# Autodesk Inventor assembly: assembly
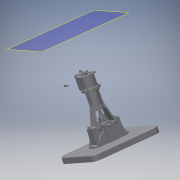
[picture p0: Inventor's stored thumbnail of the model, 180x180]
Saved by Autodesk Inventor 2017 (Build 210142000, 142)
## iProperties
Created: 2018-11-19
Part Number: assembly
Document SubType Name: Assembly
Designer: Arman Grewal
Author: Arman Grewal
## Documents named in this file (33)
- C:\Users\Arman Grewal\Desktop\Engine\assembly.iam
- C:\Users\Arman Grewal\Desktop\Engine\Piston.ipt
- C:\Users\Arman Grewal\Desktop\Engine\Piston Rod.ipt
- C:\Users\Arman Grewal\Documents\Inventor\Content Center Files\R2017\en-US\DIN 934\DIN 934 - M4 x 0.7.ipt
- C:\Users\Arman Grewal\Desktop\Engine\Crosshead.ipt
- C:\Users\Arman Grewal\Desktop\Engine\Crankrod.ipt
- C:\Users\Arman Grewal\Desktop\Engine\Crankrod Pin.ipt
- C:\Users\Arman Grewal\Desktop\Engine\Crankshaft Center Rod.ipt
- C:\Users\Arman Grewal\Desktop\Engine\Crankshaft outer rod.ipt
- C:\Users\Arman Grewal\Desktop\Engine\Crankshaft Counterweight.ipt
- C:\Users\Arman Grewal\Desktop\Engine\Vertical Steam Engine with Reverse Gear (anno 1830) Connecting Rod.ipt
- C:\Users\Arman Grewal\Desktop\Engine\Bearing Keeper.ipt
- C:\Users\Arman Grewal\Documents\Inventor\Content Center Files\R2017\en-US\DIN 84\DIN 84 - M3 x 20.ipt
- C:\Users\Arman Grewal\Desktop\Engine\Stand.ipt
- C:\Users\Arman Grewal\Desktop\Engine\Base cast f.ipt
- C:\Users\Arman Grewal\Documents\Inventor\Content Center Files\R2017\en-US\DIN 912\DIN 912 - M4 x 0.7 x 20 x 18.25.ipt
- C:\Users\Arman Grewal\Documents\Inventor\Content Center Files\R2017\en-US\DIN 6797  J\DIN 6797 - J 4.3.ipt
- C:\Users\Arman Grewal\Documents\Inventor\Content Center Files\R2017\en-US\DIN 6797  J\DIN 6797 - J 5.3.ipt
- C:\Users\Arman Grewal\Documents\Inventor\Content Center Files\R2017\en-US\DIN 934\DIN 934 - M5 x 0.8.ipt
- C:\Users\Arman Grewal\Desktop\Engine\Lower Base Bearing Holder.ipt
- C:\Users\Arman Grewal\Desktop\Engine\Upper Base Bearing Holder.ipt
- C:\Users\Arman Grewal\Documents\Inventor\Content Center Files\R2017\en-US\DIN 84\DIN 84 - M3 x 4.ipt
- C:\Users\Arman Grewal\Desktop\Engine\Standard.ipt
- C:\Users\Arman Grewal\Desktop\Engine\cylinder.ipt
- C:\Users\Arman Grewal\Documents\Inventor\Content Center Files\R2017\en-US\DIN 912\DIN 912 - M3 x 0.5 x 8 x 6.75.ipt
- C:\Users\Arman Grewal\Documents\Inventor\Content Center Files\R2017\en-US\DIN 128\DIN 128 - A3.5.ipt
- C:\Users\Arman Grewal\Desktop\Engine\Valve Plate.ipt
- C:\Users\Arman Grewal\Desktop\Engine\Steam Chest.ipt
- C:\Users\Arman Grewal\Desktop\Engine\Glands.ipt
- C:\Users\Arman Grewal\Desktop\Engine\Steam Chest Slide Valve Rod.ipt
- C:\Users\Arman Grewal\Desktop\Engine\Steam Chest Slide Valve.ipt
- C:\Users\Arman Grewal\Documents\Inventor\Content Center Files\R2017\en-US\DIN 84\DIN 84 - M2.5 x 10.ipt
- C:\Users\Arman Grewal\Documents\Inventor\Content Center Files\R2017\en-US\DIN 912\DIN 912 - M3 x 0.5 x 20 x 18.75.ipt
## Components (84 placed, 32 different names)
1. Piston:1 — Mate:1, Mate:2, Insert:1, Angle:2, Mate:56
2. Piston Rod:1 — Mate:1, Mate:2, Mate:3, Mate:4
3. DIN 934 - replaced by DIN EN 24032/28673/28674 M4:1 — Insert:1
4. Crosshead:1 — Mate:3, Mate:4, Mate:5, Mate:6
5. Crankrod:1 — Mate:5, Mate:6, Mate:7, Mate:8, Mate:9, Mate:10, Mate:11
6. Crankrod Pin:1 — Mate:7, Mate:8
7. Crankshaft Center Rod:1 — Mate:18, Mate:23, Mate:24, Mate:25, Mate:26
8. Crankshaft outer rod:1 — Mate:19, Mate:20, Mate:41
9. Crankshaft outer rod:2 — Mate:21, Mate:22
10. Vertical Steam Engine with Reverse Gear (anno 1830) Connecting Rod:1 — Mate:12, Mate:13, Mate:14, Mate:15, Mate:16, Mate:17
11. Vertical Steam Engine with Reverse Gear (anno 1830) Connecting Rod:2 — Mate:9, Mate:10, Mate:11, Mate:12, Mate:13, Mate:14, Mate:18, Mate:27
12. Bearing Keeper:1 — Mate:15, Mate:16, Mate:17, Insert:2, Insert:3
13. Crankshaft Counterweight:1 — Mate:21, Mate:22, Mate:25, Mate:26
14. Crankshaft Counterweight:2 — Mate:19, Mate:20, Mate:23, Mate:24, Mate:27, Mate:42
15. DIN 84 - replaced by DIN EN ISO 1207 M3 x 20:1 — Insert:2
16. DIN 84 - replaced by DIN EN ISO 1207 M3 x 20:2 — Insert:3
17. Stand:1 — Mate:28, Mate:29, Mate:30, Mate:32, Insert:8, Insert:9, Insert:10, Insert:11, Insert:20, Mate:36, Angle:1
18. Base cast f:1 — Mate:28, Mate:29, Mate:30, Insert:4, Insert:5, Insert:6, Insert:7, Mate:37, Flush:1, Mate:38, Mate:39, Flush:2, Mate:40, Mate:42, Mate:44, Mate:45, Mate:47, Mate:48, Mate:49, Mate:50, Mate:51, Mate:52
19. DIN 912 - replaced by DIN EN ISO 4762 M4 x 20:1 — Insert:4, Mate:31, Mate:33
20. DIN 912 - replaced by DIN EN ISO 4762 M4 x 20:2 — Insert:5
21. DIN 912 - replaced by DIN EN ISO 4762 M4 x 20:3 — Insert:6
22. DIN 912 - replaced by DIN EN ISO 4762 M4 x 20:4 — Insert:7, Mate:35
23. DIN 6797 J J 4.3:1 — Mate:31, Mate:32, Mate:34
24. DIN 6797 J J 5.3:1 — Insert:8, Insert:12, Insert:13, Insert:14, Insert:15, Insert:16, Insert:17, Insert:18, Insert:19
25. DIN 6797 J J 5.3:2 — Insert:9
26. DIN 6797 J J 5.3:3 — Insert:10
27. DIN 6797 J J 5.3:4 — Insert:11
28. DIN 934 - replaced by DIN EN 24032/28673/28674 M5:1 — Insert:12
29. DIN 934 - replaced by DIN EN 24032/28673/28674 M5:2 — Insert:13
30. DIN 934 - replaced by DIN EN 24032/28673/28674 M5:3 — Insert:14
31. DIN 934 - replaced by DIN EN 24032/28673/28674 M5:4 — Insert:15
32. DIN 934 - replaced by DIN EN 24032/28673/28674 M5:5 — Insert:16
33. DIN 934 - replaced by DIN EN 24032/28673/28674 M5:6 — Insert:17
34. DIN 934 - replaced by DIN EN 24032/28673/28674 M5:7 — Insert:18
35. DIN 934 - replaced by DIN EN 24032/28673/28674 M5:8 — Insert:19
36. DIN 934 - replaced by DIN EN 24032/28673/28674 M4:2 — Mate:33, Mate:34
37. DIN 934 - replaced by DIN EN 24032/28673/28674 M4:3 — Insert:20
38. DIN 934 - replaced by DIN EN 24032/28673/28674 M4:4 — Mate:35, Mate:36
39. Lower Base Bearing Holder:1 — Mate:37, Flush:1, Mate:38, Mate:41, Mate:46
40. Lower Base Bearing Holder:2 — Mate:39, Flush:2, Mate:40, Mate:43
41. Upper Base Bearing Holder:1 — Mate:46, Mate:47, Mate:48, Insert:21, Insert:22, Insert:23, Insert:24
42. Upper Base Bearing Holder:2 — Mate:43, Mate:44, Mate:45, Insert:25, Insert:26, Insert:27, Insert:28
43. DIN 84 - replaced by DIN EN ISO 1207 M3 x 4:1 — Insert:21
44. DIN 84 - replaced by DIN EN ISO 1207 M3 x 4:2 — Insert:22
45. DIN 84 - replaced by DIN EN ISO 1207 M3 x 4:3 — Insert:23
46. DIN 84 - replaced by DIN EN ISO 1207 M3 x 4:4 — Insert:24
47. DIN 84 - replaced by DIN EN ISO 1207 M3 x 4:5 — Insert:25
48. DIN 84 - replaced by DIN EN ISO 1207 M3 x 4:6 — Insert:26
49. DIN 84 - replaced by DIN EN ISO 1207 M3 x 4:7 — Insert:27
50. DIN 84 - replaced by DIN EN ISO 1207 M3 x 4:8 — Insert:28
51. Standard:1 — Mate:49, Mate:50, Mate:51, Mate:52, Mate:53, Mate:54, Mate:55, Insert:29, Insert:30, Insert:31, Insert:32, Insert:33, Insert:34, Insert:35, Insert:36, Insert:37, Insert:38, Insert:39, Insert:40, Insert:41, Insert:42, Insert:43, Insert:46
52. cylinder:1 — Mate:53, Angle:1, Mate:54, Mate:55, Angle:2, Mate:56, Mate:60, Mate:61, Mate:62
53. DIN 912 - replaced by DIN EN ISO 4762 M3 x 8:1 — Insert:29
54. DIN 912 - replaced by DIN EN ISO 4762 M3 x 8:2 — Insert:30
55. DIN 912 - replaced by DIN EN ISO 4762 M3 x 8:3 — Insert:31
56. DIN 912 - replaced by DIN EN ISO 4762 M3 x 8:4 — Insert:32
57. DIN 912 - replaced by DIN EN ISO 4762 M3 x 8:5 — Insert:33
58. DIN 912 - replaced by DIN EN ISO 4762 M3 x 8:6 — Insert:34
59. DIN 128 A3.5:1 — Insert:35
60. DIN 128 A3.5:2 — Insert:36, Insert:47
61. DIN 128 A3.5:3 — Insert:37, Insert:49
62. DIN 128 A3.5:4 — Insert:38, Insert:45
63. DIN 128 A3.5:5 — Insert:39, Insert:44
64. DIN 128 A3.5:6 — Insert:40, Insert:48
65. DIN 128 A3.5:7 — Insert:41, Insert:50
66. DIN 128 A3.5:8 — Insert:42
67. DIN 912 - replaced by DIN EN ISO 4762 M3 x 8:7 — Insert:43
68. DIN 912 - replaced by DIN EN ISO 4762 M3 x 8:8 — Insert:44
69. DIN 912 - replaced by DIN EN ISO 4762 M3 x 8:9 — Insert:45
70. DIN 912 - replaced by DIN EN ISO 4762 M3 x 8:10 — Insert:46
71. DIN 912 - replaced by DIN EN ISO 4762 M3 x 8:11 — Insert:47
72. DIN 912 - replaced by DIN EN ISO 4762 M3 x 8:12 — Insert:48
73. DIN 912 - replaced by DIN EN ISO 4762 M3 x 8:13 — Insert:49
74. DIN 912 - replaced by DIN EN ISO 4762 M3 x 8:14 — Insert:50
75. Valve Plate:1 — Mate:60, Mate:61, Mate:62, Mate:63, Mate:64, Mate:65
76. Steam Chest:1 — Mate:63, Mate:64, Mate:65, Mate:66, Mate:67, Mate:68, Mate:69, Mate:74
77. Glands:1 — Mate:66, Mate:67, Mate:68, Mate:69, Insert:67, Insert:68
78. Steam Chest Slide Valve Rod:1 — Mate:74, Mate:75, Mate:76, Mate:77, Mate:79
79. Steam Chest Slide Valve:1 — Mate:75, Mate:76, Mate:78, Mate:80
80. DIN 934 - replaced by DIN EN 24032/28673/28674 M4:5 — Mate:77, Mate:78
81. DIN 934 - replaced by DIN EN 24032/28673/28674 M4:6 — Mate:79, Mate:80
82. DIN 84 - replaced by DIN EN ISO 1207 M2.5 x 10:1 — Insert:67
83. DIN 84 - replaced by DIN EN ISO 1207 M2.5 x 10:2 — Insert:68
84. DIN 912 - replaced by DIN EN ISO 4762 M3 x 20:2
## Relationships (129: Mate 73, Insert 52, Flush 2, Angle 2)
- Mate:1: Piston:1 ↔ Piston Rod:1
- Mate:2: Piston:1 ↔ Piston Rod:1
- Insert:1: Piston:1 ↔ DIN 934 - replaced by DIN EN 24032/28673/28674 M4:1
- Mate:3: Piston Rod:1 ↔ Crosshead:1
- Mate:4 (-7.628 mm): Piston Rod:1 ↔ Crosshead:1
- Mate:5: Crosshead:1 ↔ Crankrod:1
- Mate:6: Crosshead:1 ↔ Crankrod:1
- Mate:7: Crankrod:1 ↔ Crankrod Pin:1
- Mate:8: Crankrod:1 ↔ Crankrod Pin:1
- Mate:9: Crankrod:1 ↔ Vertical Steam Engine with Reverse Gear (anno 1830) Connecting Rod:2
- Mate:10: Crankrod:1 ↔ Vertical Steam Engine with Reverse Gear (anno 1830) Connecting Rod:2
- Mate:11: Crankrod:1 ↔ Vertical Steam Engine with Reverse Gear (anno 1830) Connecting Rod:2
- Mate:12: Vertical Steam Engine with Reverse Gear (anno 1830) Connecting Rod:1 ↔ Vertical Steam Engine with Reverse Gear (anno 1830) Connecting Rod:2
- Mate:13: Vertical Steam Engine with Reverse Gear (anno 1830) Connecting Rod:1 ↔ Vertical Steam Engine with Reverse Gear (anno 1830) Connecting Rod:2
- Mate:14: Vertical Steam Engine with Reverse Gear (anno 1830) Connecting Rod:1 ↔ Vertical Steam Engine with Reverse Gear (anno 1830) Connecting Rod:2
- Mate:15: Vertical Steam Engine with Reverse Gear (anno 1830) Connecting Rod:1 ↔ Bearing Keeper:1
- Mate:16: Vertical Steam Engine with Reverse Gear (anno 1830) Connecting Rod:1 ↔ Bearing Keeper:1
- Mate:17: Vertical Steam Engine with Reverse Gear (anno 1830) Connecting Rod:1 ↔ Bearing Keeper:1
- Mate:18: Crankshaft Center Rod:1 ↔ Vertical Steam Engine with Reverse Gear (anno 1830) Connecting Rod:2
- Mate:19: Crankshaft outer rod:1 ↔ Crankshaft Counterweight:2
- Mate:20: Crankshaft outer rod:1 ↔ Crankshaft Counterweight:2
- Mate:21: Crankshaft outer rod:2 ↔ Crankshaft Counterweight:1
- Mate:22: Crankshaft outer rod:2 ↔ Crankshaft Counterweight:1
- Mate:23: Crankshaft Center Rod:1 ↔ Crankshaft Counterweight:2
- Mate:24: Crankshaft Center Rod:1 ↔ Crankshaft Counterweight:2
- Mate:25: Crankshaft Center Rod:1 ↔ Crankshaft Counterweight:1
- Mate:26: Crankshaft Center Rod:1 ↔ Crankshaft Counterweight:1
- Mate:27 (0.5 mm): Vertical Steam Engine with Reverse Gear (anno 1830) Connecting Rod:2 ↔ Crankshaft Counterweight:2
- Insert:2: Bearing Keeper:1 ↔ DIN 84 - replaced by DIN EN ISO 1207 M3 x 20:1
- Insert:3: Bearing Keeper:1 ↔ DIN 84 - replaced by DIN EN ISO 1207 M3 x 20:2
- Mate:28: Stand:1 ↔ Base cast f:1
- Mate:29: Stand:1 ↔ Base cast f:1
- Mate:30: Stand:1 ↔ Base cast f:1
- Insert:4: Base cast f:1 ↔ DIN 912 - replaced by DIN EN ISO 4762 M4 x 20:1
- Insert:5: Base cast f:1 ↔ DIN 912 - replaced by DIN EN ISO 4762 M4 x 20:2
- Insert:6: Base cast f:1 ↔ DIN 912 - replaced by DIN EN ISO 4762 M4 x 20:3
- Insert:7: Base cast f:1 ↔ DIN 912 - replaced by DIN EN ISO 4762 M4 x 20:4
- Mate:31: DIN 912 - replaced by DIN EN ISO 4762 M4 x 20:1 ↔ DIN 6797 J J 4.3:1
- Mate:32: Stand:1 ↔ DIN 6797 J J 4.3:1
- Insert:8: Stand:1 ↔ DIN 6797 J J 5.3:1
- Insert:9: Stand:1 ↔ DIN 6797 J J 5.3:2
- Insert:10: Stand:1 ↔ DIN 6797 J J 5.3:3
- Insert:11: Stand:1 ↔ DIN 6797 J J 5.3:4
- Insert:12: DIN 6797 J J 5.3:1 ↔ DIN 934 - replaced by DIN EN 24032/28673/28674 M5:1
- Insert:13: DIN 6797 J J 5.3:1 ↔ DIN 934 - replaced by DIN EN 24032/28673/28674 M5:2
- Insert:14: DIN 6797 J J 5.3:1 ↔ DIN 934 - replaced by DIN EN 24032/28673/28674 M5:3
- Insert:15: DIN 6797 J J 5.3:1 ↔ DIN 934 - replaced by DIN EN 24032/28673/28674 M5:4
- Insert:16: DIN 6797 J J 5.3:1 ↔ DIN 934 - replaced by DIN EN 24032/28673/28674 M5:5
- Insert:17: DIN 6797 J J 5.3:1 ↔ DIN 934 - replaced by DIN EN 24032/28673/28674 M5:6
- Insert:18: DIN 6797 J J 5.3:1 ↔ DIN 934 - replaced by DIN EN 24032/28673/28674 M5:7
- Insert:19: DIN 6797 J J 5.3:1 ↔ DIN 934 - replaced by DIN EN 24032/28673/28674 M5:8
- Mate:33: DIN 912 - replaced by DIN EN ISO 4762 M4 x 20:1 ↔ DIN 934 - replaced by DIN EN 24032/28673/28674 M4:2
- Mate:34: DIN 6797 J J 4.3:1 ↔ DIN 934 - replaced by DIN EN 24032/28673/28674 M4:2
- Insert:20: Stand:1 ↔ DIN 934 - replaced by DIN EN 24032/28673/28674 M4:3
- Mate:35: DIN 912 - replaced by DIN EN ISO 4762 M4 x 20:4 ↔ DIN 934 - replaced by DIN EN 24032/28673/28674 M4:4
- Mate:36: Stand:1 ↔ DIN 934 - replaced by DIN EN 24032/28673/28674 M4:4
- Mate:37: Base cast f:1 ↔ Lower Base Bearing Holder:1
- Flush:1: Base cast f:1 ↔ Lower Base Bearing Holder:1
- Mate:38: Base cast f:1 ↔ Lower Base Bearing Holder:1
- Mate:39: Base cast f:1 ↔ Lower Base Bearing Holder:2
- Flush:2: Base cast f:1 ↔ Lower Base Bearing Holder:2
- Mate:40: Base cast f:1 ↔ Lower Base Bearing Holder:2
- Mate:41: Crankshaft outer rod:1 ↔ Lower Base Bearing Holder:1
- Mate:42 (2.5 mm): Crankshaft Counterweight:2 ↔ Base cast f:1
- Mate:43: Lower Base Bearing Holder:2 ↔ Upper Base Bearing Holder:2
- Mate:44: Base cast f:1 ↔ Upper Base Bearing Holder:2
- Mate:45: Base cast f:1 ↔ Upper Base Bearing Holder:2
- Mate:46: Lower Base Bearing Holder:1 ↔ Upper Base Bearing Holder:1
- Mate:47: Base cast f:1 ↔ Upper Base Bearing Holder:1
- Mate:48: Base cast f:1 ↔ Upper Base Bearing Holder:1
- Insert:21: Upper Base Bearing Holder:1 ↔ DIN 84 - replaced by DIN EN ISO 1207 M3 x 4:1
- Insert:22: Upper Base Bearing Holder:1 ↔ DIN 84 - replaced by DIN EN ISO 1207 M3 x 4:2
- Insert:23: Upper Base Bearing Holder:1 ↔ DIN 84 - replaced by DIN EN ISO 1207 M3 x 4:3
- Insert:24: Upper Base Bearing Holder:1 ↔ DIN 84 - replaced by DIN EN ISO 1207 M3 x 4:4
- Insert:25: Upper Base Bearing Holder:2 ↔ DIN 84 - replaced by DIN EN ISO 1207 M3 x 4:5
- Insert:26: Upper Base Bearing Holder:2 ↔ DIN 84 - replaced by DIN EN ISO 1207 M3 x 4:6
- Insert:27: Upper Base Bearing Holder:2 ↔ DIN 84 - replaced by DIN EN ISO 1207 M3 x 4:7
- Insert:28: Upper Base Bearing Holder:2 ↔ DIN 84 - replaced by DIN EN ISO 1207 M3 x 4:8
- Mate:49: Base cast f:1 ↔ Standard:1
- Mate:50: Base cast f:1 ↔ Standard:1
- Mate:51: Base cast f:1 ↔ Standard:1
- Mate:52: Base cast f:1 ↔ Standard:1
- Mate:53: Standard:1 ↔ cylinder:1
- Angle:1 (0 deg): Stand:1 ↔ cylinder:1
- Mate:54: Standard:1 ↔ cylinder:1
- Mate:55: Standard:1 ↔ cylinder:1
- Angle:2 (0 deg): Piston:1 ↔ cylinder:1
- Mate:56: Piston:1 ↔ cylinder:1
- Insert:29: Standard:1 ↔ DIN 912 - replaced by DIN EN ISO 4762 M3 x 8:1
- Insert:30: Standard:1 ↔ DIN 912 - replaced by DIN EN ISO 4762 M3 x 8:2
- Insert:31: Standard:1 ↔ DIN 912 - replaced by DIN EN ISO 4762 M3 x 8:3
- Insert:32: Standard:1 ↔ DIN 912 - replaced by DIN EN ISO 4762 M3 x 8:4
- Insert:33: Standard:1 ↔ DIN 912 - replaced by DIN EN ISO 4762 M3 x 8:5
- Insert:34: Standard:1 ↔ DIN 912 - replaced by DIN EN ISO 4762 M3 x 8:6
- Insert:35: Standard:1 ↔ DIN 128 A3.5:1
- Insert:36: Standard:1 ↔ DIN 128 A3.5:2
- Insert:37: Standard:1 ↔ DIN 128 A3.5:3
- Insert:38: Standard:1 ↔ DIN 128 A3.5:4
- Insert:39: Standard:1 ↔ DIN 128 A3.5:5
- Insert:40: Standard:1 ↔ DIN 128 A3.5:6
- Insert:41: Standard:1 ↔ DIN 128 A3.5:7
- Insert:42: Standard:1 ↔ DIN 128 A3.5:8
- Insert:43: Standard:1 ↔ DIN 912 - replaced by DIN EN ISO 4762 M3 x 8:7
- Insert:44: DIN 128 A3.5:5 ↔ DIN 912 - replaced by DIN EN ISO 4762 M3 x 8:8
- Insert:45: DIN 128 A3.5:4 ↔ DIN 912 - replaced by DIN EN ISO 4762 M3 x 8:9
- Insert:46: Standard:1 ↔ DIN 912 - replaced by DIN EN ISO 4762 M3 x 8:10
- Insert:47: DIN 128 A3.5:2 ↔ DIN 912 - replaced by DIN EN ISO 4762 M3 x 8:11
- Insert:48: DIN 128 A3.5:6 ↔ DIN 912 - replaced by DIN EN ISO 4762 M3 x 8:12
- Insert:49: DIN 128 A3.5:3 ↔ DIN 912 - replaced by DIN EN ISO 4762 M3 x 8:13
- Insert:50: DIN 128 A3.5:7 ↔ DIN 912 - replaced by DIN EN ISO 4762 M3 x 8:14
- Mate:60: cylinder:1 ↔ Valve Plate:1
- Mate:61: cylinder:1 ↔ Valve Plate:1
- Mate:62: cylinder:1 ↔ Valve Plate:1
- Mate:63: Valve Plate:1 ↔ Steam Chest:1
- Mate:64: Valve Plate:1 ↔ Steam Chest:1
- Mate:65: Valve Plate:1 ↔ Steam Chest:1
- Mate:66: Steam Chest:1 ↔ Glands:1
- Mate:67: Steam Chest:1 ↔ Glands:1
- Mate:68: Steam Chest:1 ↔ Glands:1
- Mate:69: Steam Chest:1 ↔ Glands:1
- Mate:74: Steam Chest:1 ↔ Steam Chest Slide Valve Rod:1
- Mate:75 (2.844 mm): Steam Chest Slide Valve Rod:1 ↔ Steam Chest Slide Valve:1
- Mate:76: Steam Chest Slide Valve Rod:1 ↔ Steam Chest Slide Valve:1
- Mate:77: Steam Chest Slide Valve Rod:1 ↔ DIN 934 - replaced by DIN EN 24032/28673/28674 M4:5
- Mate:78: Steam Chest Slide Valve:1 ↔ DIN 934 - replaced by DIN EN 24032/28673/28674 M4:5
- Mate:79: Steam Chest Slide Valve Rod:1 ↔ DIN 934 - replaced by DIN EN 24032/28673/28674 M4:6
- Mate:80: Steam Chest Slide Valve:1 ↔ DIN 934 - replaced by DIN EN 24032/28673/28674 M4:6
- Insert:67: Glands:1 ↔ DIN 84 - replaced by DIN EN ISO 1207 M2.5 x 10:1
- Insert:68: Glands:1 ↔ DIN 84 - replaced by DIN EN ISO 1207 M2.5 x 10:2
